# Autodesk Inventor assembly: chassis
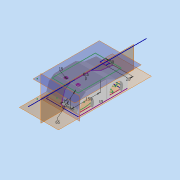
[picture p0: Inventor's stored thumbnail of the model, 180x180]
Saved by Autodesk Inventor 2022 (Build 260153000, 153)
## iProperties
Created: 2021-06-06
Part Number: chassis
Document SubType Name: Assembly
Designer: Default
Author: Default
## Documents named in this file (4)
- E:\source\repos\S21\fachübergreifend\fennec bot\fennec-jet-racer\Konstruktion\chassis.iam
- E:\source\repos\S21\fachübergreifend\fennec bot\fennec-jet-racer\Konstruktion\struktur.ipt
- E:\source\repos\S21\fachübergreifend\fennec bot\fennec-jet-racer\Konstruktion\chassis_front.ipt
- E:\source\repos\S21\fachübergreifend\fennec bot\fennec-jet-racer\Konstruktion\chassis_back.ipt
## Components (3 placed, 3 different names)
1. struktur:1 — Passend:1, Passend:2, Passend:3, Passend:4
2. chassis_front:1 — Passend:2, Passend:3
3. chassis_back:1
## Relationships (4: Mate 4)
- Passend:1 [Mate]: struktur:1
- Passend:2 [Mate]: struktur:1 ↔ chassis_front:1
- Passend:3 [Mate]: struktur:1 ↔ chassis_front:1
- Passend:4 [Mate]: struktur:1
